# Autodesk Inventor assembly: Assembly2
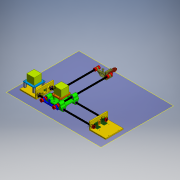
[picture p0: Inventor's stored thumbnail of the model, 180x180]
Saved by Autodesk Inventor 2016 (Build 200138000, 138)
## iProperties
Created: 2018-01-17
Part Number: Assembly2
Document SubType Name: Assembly
Designer: student
Author: student
## Documents named in this file (16)
- C:\gitHub_projects\Plotter_CAD\plotter_project\PLOTTER\Assembly2.iam
- C:\gitHub_projects\Plotter_CAD\plotter_project\PLOTTER\Part2.ipt
- C:\gitHub_projects\Plotter_CAD\plotter_project\PLOTTER\axis plotter motor timing pulley.ipt
- C:\gitHub_projects\Plotter_CAD\plotter_project\PLOTTER\Part3.ipt
- C:\gitHub_projects\Plotter_CAD\plotter_project\PLOTTER\Part9.ipt
- C:\gitHub_projects\Plotter_CAD\plotter_project\PLOTTER\Part14.ipt
- C:\gitHub_projects\Plotter_CAD\plotter_project\PLOTTER\Part15.ipt
- C:\gitHub_projects\Plotter_CAD\plotter_project\PLOTTER\Part16.ipt
- C:\gitHub_projects\Plotter_CAD\plotter_project\PLOTTER\Part10.ipt
- C:\gitHub_projects\Plotter_CAD\plotter_project\PLOTTER\rod.ipt
- C:\gitHub_projects\Plotter_CAD\plotter_project\PLOTTER\axis plotter berring mount.ipt
- C:\gitHub_projects\Plotter_CAD\plotter_project\PLOTTER\Part1.ipt
- C:\gitHub_projects\Plotter_CAD\plotter_project\PLOTTER\Part4.ipt
- C:\gitHub_projects\Plotter_CAD\plotter_project\PLOTTER\axis plotter. y axis.ipt
- C:\gitHub_projects\Plotter_CAD\plotter_project\PLOTTER\PEN MOUNT ORIGINAL_copy.ipt
- C:\gitHub_projects\Plotter_CAD\plotter_project\PLOTTER\pen_holder_2.ipt
## Components (47 placed, 15 different names)
1. Part2:1 — Insert:1, Angle:3, Mate:1, Mate:2, Angle:5, Angle:10
2. axis plotter motor timing pulley:1 — Insert:1
3. Part3:1 — Mate:1, Mate:2, Rigid:1, Rigid:4, Angle:4, Flush:2, Rigid:5, Rigid:6
4. Part9:1 — Rigid:1
5. Part9:3 — Rigid:4
6. Part9:4 — Rigid:5
7. Part9:5 — Rigid:6, Flush:3
8. Part14:1 — Flush:3, Flush:4, Mate:5, Mate:8
9. Part15:1 — Flush:4, Mate:3, Mate:4, Mate:6, Mate:7, Rigid:9, Rigid:10
10. Part16:1 — Mate:3, Mate:4, Mate:5
11. Part16:2 — Mate:6, Mate:7, Mate:8
12. Part10:1 — Rigid:7, Rigid:10
13. rod:1 — Rigid:7, Rigid:11, Mate:19, Mate:23, Cylindrical:1
14. rod:2 — Rigid:8, Rigid:12, Mate:21, Mate:22
15. Part10:2 — Rigid:8, Rigid:9
16. axis plotter berring mount:1 — Rigid:13, Rigid:14, Rigid:15, Rigid:16, Rigid:17, Rigid:18, Rigid:19, Rigid:20, Cylindrical:1, Rigid:21, Mate:25, Mate:26, Cylindrical:2
17. Part1:1 — Rigid:14, Mate:22
18. Part14:2 — Mate:14, Mate:15, Mate:16, Mate:17, Mate:18, Angle:11
19. Part15:2 — Mate:14, Mate:15, Mate:16, Mate:19, Mate:20, Mate:21, Rigid:25
20. Part16:3 — Mate:18
21. Part16:4 — Mate:17
22. Part10:3 — Rigid:12
23. Part10:4 — Rigid:11, Mate:20
24. Part1:2 — Rigid:13, Mate:23
25. Part1:3 — Rigid:19
26. Part1:4 — Rigid:20
27. Part1:5 — Rigid:18
28. Part1:6 — Rigid:17
29. Part1:7 — Rigid:16
30. Part1:8 — Rigid:15
31. Part4:1 — Rigid:21, Rigid:24
32. rod:3 — Rigid:23, Mate:26, Mate:27, Rigid:28
33. rod:4 — Rigid:22, Mate:25, Mate:28, Rigid:29
34. Part10:5 — Rigid:23, Rigid:27
35. Part10:6 — Rigid:22, Rigid:26
36. Part2:2 — Rigid:24, Rotational:1
37. axis plotter motor timing pulley:2 — Rotational:1
38. axis plotter motor timing pulley:3 — Rigid:25
39. axis plotter. y axis:1 — Rigid:26, Rigid:27, Cylindrical:2, Rigid:32, Rigid:33
40. PEN MOUNT ORIGINAL_copy:1 — Mate:27, Mate:28, Mate:29, Rigid:30, Rigid:31, Slider:1
41. Part10:7 — Rigid:29
42. Part10:8 — Rigid:31
43. Part10:9 — Rigid:30
44. Part10:10 — Rigid:28, Mate:29
45. Part10:11 — Rigid:33
46. Part10:12 — Rigid:32
47. pen_holder_2:1 — Slider:1
## Relationships (74: WeldJoint 31, Mate 27, Angle 7, Flush 4, CylindricalJoint 2, Insert 1, RevoluteJoint 1, TranslationJoint 1)
- Insert:1: Part2:1 ↔ axis plotter motor timing pulley:1
- Angle:3 (180 deg): Part2:1
- Mate:1: Part2:1 ↔ Part3:1
- Mate:2: Part2:1 ↔ Part3:1
- Rigid:1 [WeldJoint]: Part3:1 ↔ Part9:1
- Rigid:4 [WeldJoint]: Part3:1 ↔ Part9:3
- Angle:4 (0 deg): Part3:1
- Flush:1 (-56 mm)
- Angle:5 (0 deg): Part2:1
- Flush:2 (30 mm): Part3:1
- Angle:8 (0 deg)
- Angle:9 (0 deg)
- Rigid:5 [WeldJoint]: Part3:1 ↔ Part9:4
- Rigid:6 [WeldJoint]: Part3:1 ↔ Part9:5
- Flush:3: Part9:5 ↔ Part14:1
- Flush:4: Part14:1 ↔ Part15:1
- Angle:10 (0 deg): Part2:1
- Mate:3: Part15:1 ↔ Part16:1
- Mate:4: Part15:1 ↔ Part16:1
- Mate:5: Part14:1 ↔ Part16:1
- Mate:6: Part15:1 ↔ Part16:2
- Mate:7: Part15:1 ↔ Part16:2
- Mate:8: Part14:1 ↔ Part16:2
- Rigid:7 [WeldJoint]: Part10:1 ↔ rod:1
- Rigid:8 [WeldJoint]: rod:2 ↔ Part10:2
- Rigid:9 [WeldJoint]: Part15:1 ↔ Part10:2
- Rigid:10 [WeldJoint]: Part15:1 ↔ Part10:1
- [Mate]: Part15:2 ↔ Part16:3
- [Mate]: Part15:2 ↔ Part16:3
- [Mate]: Part15:2 ↔ Part16:4
- [Mate]: Part15:2 ↔ Part16:4
- Mate:14: Part14:2 ↔ Part15:2
- Mate:15: Part14:2 ↔ Part15:2
- Mate:16: Part14:2 ↔ Part15:2
- Mate:17: Part14:2 ↔ Part16:4
- Mate:18: Part14:2 ↔ Part16:3
- Angle:11 (180 deg): Part14:2
- Rigid:11 [WeldJoint]: rod:1 ↔ Part10:4
- Rigid:12 [WeldJoint]: rod:2 ↔ Part10:3
- Mate:19: rod:1 ↔ Part15:2
- Mate:20: Part15:2 ↔ Part10:4
- Mate:21: rod:2 ↔ Part15:2
- Rigid:13 [WeldJoint]: axis plotter berring mount:1 ↔ Part1:2
- Rigid:14 [WeldJoint]: axis plotter berring mount:1 ↔ Part1:1
- Rigid:15 [WeldJoint]: axis plotter berring mount:1 ↔ Part1:8
- Rigid:16 [WeldJoint]: axis plotter berring mount:1 ↔ Part1:7
- Rigid:17 [WeldJoint]: axis plotter berring mount:1 ↔ Part1:6
- Rigid:18 [WeldJoint]: axis plotter berring mount:1 ↔ Part1:5
- Rigid:19 [WeldJoint]: axis plotter berring mount:1 ↔ Part1:3
- Rigid:20 [WeldJoint]: axis plotter berring mount:1 ↔ Part1:4
- Mate:22: rod:2 ↔ Part1:1
- Mate:23: rod:1 ↔ Part1:2
- Cylindrical:1: rod:1 ↔ axis plotter berring mount:1
- Rigid:21 [WeldJoint]: axis plotter berring mount:1 ↔ Part4:1
- Rigid:22 [WeldJoint]: rod:4 ↔ Part10:6
- Rigid:23 [WeldJoint]: rod:3 ↔ Part10:5
- Rigid:24 [WeldJoint]: Part4:1 ↔ Part2:2
- Rotational:1 [RevoluteJoint]: Part2:2 ↔ axis plotter motor timing pulley:2
- Rigid:25 [WeldJoint]: Part15:2 ↔ axis plotter motor timing pulley:3
- Mate:25: axis plotter berring mount:1 ↔ rod:4
- Rigid:26 [WeldJoint]: Part10:6 ↔ axis plotter. y axis:1
- Rigid:27 [WeldJoint]: Part10:5 ↔ axis plotter. y axis:1
- Mate:26: axis plotter berring mount:1 ↔ rod:3
- Cylindrical:2: axis plotter berring mount:1 ↔ axis plotter. y axis:1
- Mate:27: rod:3 ↔ PEN MOUNT ORIGINAL_copy:1
- Mate:28: rod:4 ↔ PEN MOUNT ORIGINAL_copy:1
- Rigid:28 [WeldJoint]: rod:3 ↔ Part10:10
- Rigid:29 [WeldJoint]: rod:4 ↔ Part10:7
- Mate:29: PEN MOUNT ORIGINAL_copy:1 ↔ Part10:10
- Rigid:30 [WeldJoint]: PEN MOUNT ORIGINAL_copy:1 ↔ Part10:9
- Rigid:31 [WeldJoint]: PEN MOUNT ORIGINAL_copy:1 ↔ Part10:8
- Rigid:32 [WeldJoint]: axis plotter. y axis:1 ↔ Part10:12
- Rigid:33 [WeldJoint]: axis plotter. y axis:1 ↔ Part10:11
- Slider:1 [TranslationJoint]: PEN MOUNT ORIGINAL_copy:1 ↔ pen_holder_2:1
## Named parameters: d73_d62 = 0 mm, d74_d63 = 0 mm, d76_d65 = 0 mm, d77_d66 = 0 mm
